# Autodesk Inventor assembly: steering_kingpin_left_assy
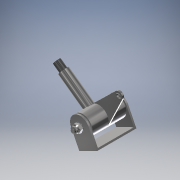
[picture p0: Inventor's stored thumbnail of the model, 180x180]
Saved by Autodesk Inventor 2019 (Build 230136000, 136)
## iProperties
Created: 2019-04-24
Part Number: steering_kingpin_left_assy
Document SubType Name: Assembly
Designer: callum.snowden
Mass: 517.605 g
Surface Area: 457.609 cm^2
Volume: 65.937 cm^3
Density: 7.85 g/cm^3
Author: callum.snowden
## Documents named in this file (9)
- C:\Users\callum.snowden\Documents\GitHub\clasohlsonkart\mechanical\frame\steering_kingpin_left_assy.iam
- C:\Users\callum.snowden\Documents\GitHub\clasohlsonkart\mechanical\frame\steering_kingpin_left.ipt
- C:\Users\callum.snowden\Documents\Inventor\Content Center Files\R2019\en-US\SKF 2Z - with two shields\SKF 2Z6200-2Z.ipt
- C:\Users\callum.snowden\Documents\GitHub\clasohlsonkart\mechanical\frame\steering_kingpin_bearing_spacer.ipt
- C:\Users\callum.snowden\Documents\GitHub\clasohlsonkart\mechanical\frame\steering_kingpin_bracket.ipt
- C:\Users\callum.snowden\Documents\Inventor\Content Center Files\R2019\en-US\BS 4320(2)\BS 4320 - M10 (Form A).ipt
- C:\Users\callum.snowden\Documents\Inventor\Content Center Files\R2019\en-US\BS 4168(7)\BS 4168 - 10 x 70.ipt
- C:\Users\callum.snowden\Documents\Inventor\Content Center Files\R2019\en-US\DIN 6797  A\DIN 6797 - A 8.4.ipt
- C:\Users\callum.snowden\Documents\Inventor\Content Center Files\R2019\en-US\ANSI B18.16.3M(2)\ANSI B18.16.3M - Property Class 5 and 10 - Metric M8 x 1.25 Top Insert Type.ipt
## Components (10 placed, 8 different names)
1. steering_kingpin_left:1 — Rigid:1, Rigid:3
2. SKF 2Z- with two shields SKF 2Z6200-2Z:1 — Rigid:3, Mate:1
3. SKF 2Z- with two shields SKF 2Z6200-2Z:2 — Rigid:1, Rigid:2, Mate:2
4. steering_kingpin_bearing_spacer:1 — Rigid:2
5. steering_kingpin_bracket:1 — Rotational:1, Mate:3, Rotational:2
6. BS 4320 Form AB M10 (Form A):1 — Mate:1, Rotational:1
7. BS 4320 Form AB M10 (Form A):2 — Mate:2, Mate:3
8. BS 4168 : Part 7 Hexagon socket screws and wrench keys, metric series- Specification for hexagon socket shoulder screws - Metric 10 x 70:1 — Rotational:2, Rotational:3
9. DIN 6797 A A 8.4:1 — Rotational:3, Rigid:4
10. Prevailing Torque Type Hex Nut - Steel Metric Property Class 5 and 10 - Metric M8 x 1.25 Top Insert Type:1 — Rigid:4
## Relationships (10: WeldJoint 4, Mate 3, RevoluteJoint 3)
- Rigid:1 [WeldJoint]: steering_kingpin_left:1 ↔ SKF 2Z- with two shields SKF 2Z6200-2Z:2
- Rigid:2 [WeldJoint]: SKF 2Z- with two shields SKF 2Z6200-2Z:2 ↔ steering_kingpin_bearing_spacer:1
- Rigid:3 [WeldJoint]: steering_kingpin_left:1 ↔ SKF 2Z- with two shields SKF 2Z6200-2Z:1
- Mate:1: SKF 2Z- with two shields SKF 2Z6200-2Z:1 ↔ BS 4320 Form AB M10 (Form A):1
- Mate:2: SKF 2Z- with two shields SKF 2Z6200-2Z:2 ↔ BS 4320 Form AB M10 (Form A):2
- Rotational:1 [RevoluteJoint]: steering_kingpin_bracket:1 ↔ BS 4320 Form AB M10 (Form A):1
- Mate:3: steering_kingpin_bracket:1 ↔ BS 4320 Form AB M10 (Form A):2
- Rotational:2 [RevoluteJoint]: steering_kingpin_bracket:1 ↔ BS 4168 : Part 7 Hexagon socket screws and wrench keys, metric series- Specification for hexagon socket shoulder screws - Metric 10 x 70:1
- Rotational:3 [RevoluteJoint]: BS 4168 : Part 7 Hexagon socket screws and wrench keys, metric series- Specification for hexagon socket shoulder screws - Metric 10 x 70:1 ↔ DIN 6797 A A 8.4:1
- Rigid:4 [WeldJoint]: DIN 6797 A A 8.4:1 ↔ Prevailing Torque Type Hex Nut - Steel Metric Property Class 5 and 10 - Metric M8 x 1.25 Top Insert Type:1
